# Autodesk Inventor assembly: BallBot
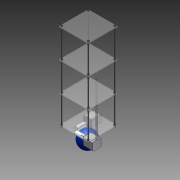
[picture p0: Inventor's stored thumbnail of the model, 180x180]
Saved by Autodesk Inventor 2012 (Build 160160000, 160)
## iProperties
Created: 2012-10-02
Part Number: BallBot
Document SubType Name: Assembly
Designer: agmlego
Author: agmlego
## Documents named in this file (8)
- C:\Users\Andrew G. Meyer\Documents\Projects\BallBot\Little\CAD\BallBot.iam
- C:\Users\Andrew G. Meyer\Documents\Projects\BallBot\Little\CAD\Platform.ipt
- C:\Users\Andrew G. Meyer\Documents\Projects\BallBot\Little\CAD\Rod.ipt
- C:\Users\Andrew G. Meyer\Documents\Projects\BallBot\Little\CAD\Ball.ipt
- C:\Users\Andrew G. Meyer\Documents\Inventor\Content Center Files\R2012\en-US\ANSI B 18.2.4.1 M(1)\ANSI B 18.2.4.1 M - M3 x 0.5Style 1.ipt
- C:\Users\Andrew G. Meyer\Documents\Projects\BallBot\Little\CAD\211-13-01.ipt
- C:\Users\Andrew G. Meyer\Documents\Projects\BallBot\Little\CAD\Roller.ipt
- C:\Users\Andrew G. Meyer\Documents\Inventor\Content Center Files\R2012\en-US\ANSI B18.3(08)\ANSI B18.3 - 4-48 UNF - 0.125(24).ipt
## Components (49 placed, 7 different names)
1. Platform:1 — Mate:50, Mate:51, Mate:53, Mate:55, Mate:80, Mate:81, Mate:82, Mate:83, Mate:84, Mate:85, Mate:86, Mate:87, Mate:95, Mate:96, Flush:9, Flush:10, Tangent:7, Flush:11, Flush:12
2. Platform:2 — Mate:34, Mate:35, Mate:36, Mate:37, Mate:56, Mate:57, Mate:58, Mate:59, Mate:60, Mate:61, Mate:62, Mate:63, Mate:89
3. Platform:3 — Mate:38, Mate:39, Mate:40, Mate:41, Mate:43, Mate:44, Mate:45, Mate:72, Mate:73, Mate:74, Mate:75, Mate:76, Mate:77, Mate:78, Mate:79, Mate:88
4. Platform:4 — Mate:42, Mate:64, Mate:65, Mate:66, Mate:67, Mate:68, Mate:69, Mate:70, Mate:71, Mate:88, Mate:89, Mate:90
5. Rod:1 — Mate:4, Mate:5, Mate:6, Mate:7, Mate:8, Mate:9, Mate:10, Mate:11, Mate:34, Mate:38, Mate:42, Mate:84, Flush:4, Flush:6
6. Rod:2 — Mate:1, Mate:3, Mate:12, Mate:13, Mate:14, Mate:15, Mate:16, Mate:17, Mate:35, Mate:39, Mate:43, Mate:80, Flush:1, Flush:5
7. Rod:3 — Mate:18, Mate:19, Mate:20, Mate:21, Mate:22, Mate:23, Mate:24, Mate:25, Mate:36, Mate:40, Mate:44, Mate:82, Flush:2, Flush:8, Mate:90
8. Rod:4 — Mate:26, Mate:27, Mate:28, Mate:29, Mate:30, Mate:31, Mate:32, Mate:33, Mate:37, Mate:41, Mate:45, Mate:86, Flush:3, Flush:7
9. Ball:1 — Tangent:5, Tangent:6, Tangent:7
10. Hex Nut Metric M3 x 0.5:1 — Mate:26, Mate:87, Flush:3
11. Hex Nut Metric M3 x 0.5:2 — Mate:27, Mate:55
12. Hex Nut Metric M3 x 0.5:3 — Mate:28, Mate:67
13. Hex Nut Metric M3 x 0.5:4 — Mate:29, Mate:63
14. Hex Nut Metric M3 x 0.5:5 — Mate:30, Mate:58
15. Hex Nut Metric M3 x 0.5:6 — Mate:31, Mate:78, Flush:7
16. Hex Nut Metric M3 x 0.5:7 — Mate:32, Mate:70
17. Hex Nut Metric M3 x 0.5:8 — Mate:33, Mate:74
18. Hex Nut Metric M3 x 0.5:9 — Mate:4, Mate:66
19. Hex Nut Metric M3 x 0.5:10 — Mate:5, Mate:57
20. Hex Nut Metric M3 x 0.5:11 — Mate:6, Mate:85, Flush:4
21. Hex Nut Metric M3 x 0.5:12 — Mate:7, Mate:53
22. Hex Nut Metric M3 x 0.5:13 — Mate:8, Mate:71
23. Hex Nut Metric M3 x 0.5:14 — Mate:9, Mate:75
24. Hex Nut Metric M3 x 0.5:15 — Mate:10, Mate:79, Flush:6
25. Hex Nut Metric M3 x 0.5:16 — Mate:11, Mate:62
26. Hex Nut Metric M3 x 0.5:17 — Mate:1, Mate:81, Flush:1
27. Hex Nut Metric M3 x 0.5:18 — Mate:3, Mate:51
28. Hex Nut Metric M3 x 0.5:19 — Mate:12, Mate:73
29. Hex Nut Metric M3 x 0.5:20 — Mate:13, Mate:56
30. Hex Nut Metric M3 x 0.5:21 — Mate:14, Mate:65
31. Hex Nut Metric M3 x 0.5:22 — Mate:15, Mate:69
32. Hex Nut Metric M3 x 0.5:23 — Mate:16, Mate:61
33. Hex Nut Metric M3 x 0.5:24 — Mate:17, Mate:77, Flush:5
34. Hex Nut Metric M3 x 0.5:25 — Mate:18, Mate:50
35. Hex Nut Metric M3 x 0.5:26 — Mate:19, Mate:60
36. Hex Nut Metric M3 x 0.5:27 — Mate:20, Mate:59
37. Hex Nut Metric M3 x 0.5:28 — Mate:21, Mate:68
38. Hex Nut Metric M3 x 0.5:29 — Mate:22, Mate:83, Flush:2
39. Hex Nut Metric M3 x 0.5:30 — Mate:23, Mate:76, Flush:8
40. Hex Nut Metric M3 x 0.5:31 — Mate:24, Mate:72
41. Hex Nut Metric M3 x 0.5:32 — Mate:25, Mate:64
42. 211-13-01:1 — Insert:1, Tangent:3, Tangent:4, Mate:95, Flush:10, Flush:11
43. 211-13-01:3 — Insert:2, Tangent:1, Tangent:2, Mate:96, Flush:9, Flush:12
44. Roller:1 — Insert:2, Mate:91, Mate:92, Tangent:6
45. Roller:2 — Insert:1, Mate:93, Mate:94, Tangent:5
46. Hexagon Socket Set Screw - Flat Point - Inch 4-48 UNF x 0.125:3 — Mate:91, Tangent:1
47. Hexagon Socket Set Screw - Flat Point - Inch 4-48 UNF x 0.125:1 — Mate:94, Tangent:4
48. Hexagon Socket Set Screw - Flat Point - Inch 4-48 UNF x 0.125:4 — Mate:92, Tangent:2
49. Hexagon Socket Set Screw - Flat Point - Inch 4-48 UNF x 0.125:2 — Mate:93, Tangent:3
## Relationships (110: Mate 89, Flush 12, Tangent 7, Insert 2)
- Mate:1: Rod:2 ↔ Hex Nut Metric M3 x 0.5:17
- Mate:3: Rod:2 ↔ Hex Nut Metric M3 x 0.5:18
- Mate:4: Rod:1 ↔ Hex Nut Metric M3 x 0.5:9
- Mate:5: Rod:1 ↔ Hex Nut Metric M3 x 0.5:10
- Mate:6: Rod:1 ↔ Hex Nut Metric M3 x 0.5:11
- Mate:7: Rod:1 ↔ Hex Nut Metric M3 x 0.5:12
- Mate:8: Rod:1 ↔ Hex Nut Metric M3 x 0.5:13
- Mate:9: Rod:1 ↔ Hex Nut Metric M3 x 0.5:14
- Mate:10: Rod:1 ↔ Hex Nut Metric M3 x 0.5:15
- Mate:11: Rod:1 ↔ Hex Nut Metric M3 x 0.5:16
- Mate:12: Rod:2 ↔ Hex Nut Metric M3 x 0.5:19
- Mate:13: Rod:2 ↔ Hex Nut Metric M3 x 0.5:20
- Mate:14: Rod:2 ↔ Hex Nut Metric M3 x 0.5:21
- Mate:15: Rod:2 ↔ Hex Nut Metric M3 x 0.5:22
- Mate:16: Rod:2 ↔ Hex Nut Metric M3 x 0.5:23
- Mate:17: Rod:2 ↔ Hex Nut Metric M3 x 0.5:24
- Mate:18: Rod:3 ↔ Hex Nut Metric M3 x 0.5:25
- Mate:19: Rod:3 ↔ Hex Nut Metric M3 x 0.5:26
- Mate:20: Rod:3 ↔ Hex Nut Metric M3 x 0.5:27
- Mate:21: Rod:3 ↔ Hex Nut Metric M3 x 0.5:28
- Mate:22: Rod:3 ↔ Hex Nut Metric M3 x 0.5:29
- Mate:23: Rod:3 ↔ Hex Nut Metric M3 x 0.5:30
- Mate:24: Rod:3 ↔ Hex Nut Metric M3 x 0.5:31
- Mate:25: Rod:3 ↔ Hex Nut Metric M3 x 0.5:32
- Mate:26: Rod:4 ↔ Hex Nut Metric M3 x 0.5:1
- Mate:27: Rod:4 ↔ Hex Nut Metric M3 x 0.5:2
- Mate:28: Rod:4 ↔ Hex Nut Metric M3 x 0.5:3
- Mate:29: Rod:4 ↔ Hex Nut Metric M3 x 0.5:4
- Mate:30: Rod:4 ↔ Hex Nut Metric M3 x 0.5:5
- Mate:31: Rod:4 ↔ Hex Nut Metric M3 x 0.5:6
- Mate:32: Rod:4 ↔ Hex Nut Metric M3 x 0.5:7
- Mate:33: Rod:4 ↔ Hex Nut Metric M3 x 0.5:8
- Mate:34: Platform:2 ↔ Rod:1
- Mate:35: Platform:2 ↔ Rod:2
- Mate:36: Platform:2 ↔ Rod:3
- Mate:37: Platform:2 ↔ Rod:4
- Mate:38: Platform:3 ↔ Rod:1
- Mate:39: Platform:3 ↔ Rod:2
- Mate:40: Platform:3 ↔ Rod:3
- Mate:41: Platform:3 ↔ Rod:4
- Mate:42: Platform:4 ↔ Rod:1
- Mate:43: Platform:3 ↔ Rod:2
- Mate:44: Platform:3 ↔ Rod:3
- Mate:45: Platform:3 ↔ Rod:4
- Mate:50: Platform:1 ↔ Hex Nut Metric M3 x 0.5:25
- Mate:51: Platform:1 ↔ Hex Nut Metric M3 x 0.5:18
- Mate:53: Platform:1 ↔ Hex Nut Metric M3 x 0.5:12
- Mate:55: Platform:1 ↔ Hex Nut Metric M3 x 0.5:2
- Mate:56: Platform:2 ↔ Hex Nut Metric M3 x 0.5:20
- Mate:57: Platform:2 ↔ Hex Nut Metric M3 x 0.5:10
- Mate:58: Platform:2 ↔ Hex Nut Metric M3 x 0.5:5
- Mate:59: Platform:2 ↔ Hex Nut Metric M3 x 0.5:27
- Mate:60: Platform:2 ↔ Hex Nut Metric M3 x 0.5:26
- Mate:61: Platform:2 ↔ Hex Nut Metric M3 x 0.5:23
- Mate:62: Platform:2 ↔ Hex Nut Metric M3 x 0.5:16
- Mate:63: Platform:2 ↔ Hex Nut Metric M3 x 0.5:4
- Mate:64: Platform:4 ↔ Hex Nut Metric M3 x 0.5:32
- Mate:65: Platform:4 ↔ Hex Nut Metric M3 x 0.5:21
- Mate:66: Platform:4 ↔ Hex Nut Metric M3 x 0.5:9
- Mate:67: Platform:4 ↔ Hex Nut Metric M3 x 0.5:3
- Mate:68: Platform:4 ↔ Hex Nut Metric M3 x 0.5:28
- Mate:69: Platform:4 ↔ Hex Nut Metric M3 x 0.5:22
- Mate:70: Platform:4 ↔ Hex Nut Metric M3 x 0.5:7
- Mate:71: Platform:4 ↔ Hex Nut Metric M3 x 0.5:13
- Mate:72: Platform:3 ↔ Hex Nut Metric M3 x 0.5:31
- Mate:73: Platform:3 ↔ Hex Nut Metric M3 x 0.5:19
- Mate:74: Platform:3 ↔ Hex Nut Metric M3 x 0.5:8
- Mate:75: Platform:3 ↔ Hex Nut Metric M3 x 0.5:14
- Mate:76: Platform:3 ↔ Hex Nut Metric M3 x 0.5:30
- Mate:77: Platform:3 ↔ Hex Nut Metric M3 x 0.5:24
- Mate:78: Platform:3 ↔ Hex Nut Metric M3 x 0.5:6
- Mate:79: Platform:3 ↔ Hex Nut Metric M3 x 0.5:15
- Mate:80: Platform:1 ↔ Rod:2
- Mate:81: Platform:1 ↔ Hex Nut Metric M3 x 0.5:17
- Mate:82: Platform:1 ↔ Rod:3
- Mate:83: Platform:1 ↔ Hex Nut Metric M3 x 0.5:29
- Mate:84: Platform:1 ↔ Rod:1
- Mate:85: Platform:1 ↔ Hex Nut Metric M3 x 0.5:11
- Mate:86: Platform:1 ↔ Rod:4
- Mate:87: Platform:1 ↔ Hex Nut Metric M3 x 0.5:1
- Flush:1 (-1 mm): Rod:2 ↔ Hex Nut Metric M3 x 0.5:17
- Flush:2 (-1 mm): Rod:3 ↔ Hex Nut Metric M3 x 0.5:29
- Flush:3 (-1 mm): Rod:4 ↔ Hex Nut Metric M3 x 0.5:1
- Flush:4 (-1 mm): Rod:1 ↔ Hex Nut Metric M3 x 0.5:11
- Flush:5 (-1 mm): Rod:2 ↔ Hex Nut Metric M3 x 0.5:24
- Flush:6 (-1 mm): Rod:1 ↔ Hex Nut Metric M3 x 0.5:15
- Flush:7 (-1 mm): Rod:4 ↔ Hex Nut Metric M3 x 0.5:6
- Flush:8 (-1 mm): Rod:3 ↔ Hex Nut Metric M3 x 0.5:30
- Mate:88 (95 mm): Platform:3 ↔ Platform:4
- Mate:89 (95 mm): Platform:2 ↔ Platform:4
- Mate:90: Platform:4 ↔ Rod:3
- Insert:1: 211-13-01:1 ↔ Roller:2
- Insert:2: 211-13-01:3 ↔ Roller:1
- Mate:91: Roller:1 ↔ Hexagon Socket Set Screw - Flat Point - Inch 4-48 UNF x 0.125:3
- Mate:92: Roller:1 ↔ Hexagon Socket Set Screw - Flat Point - Inch 4-48 UNF x 0.125:4
- Mate:93: Roller:2 ↔ Hexagon Socket Set Screw - Flat Point - Inch 4-48 UNF x 0.125:2
- Mate:94: Roller:2 ↔ Hexagon Socket Set Screw - Flat Point - Inch 4-48 UNF x 0.125:1
- Tangent:1: 211-13-01:3 ↔ Hexagon Socket Set Screw - Flat Point - Inch 4-48 UNF x 0.125:3
- Tangent:2: 211-13-01:3 ↔ Hexagon Socket Set Screw - Flat Point - Inch 4-48 UNF x 0.125:4
- Tangent:3: 211-13-01:1 ↔ Hexagon Socket Set Screw - Flat Point - Inch 4-48 UNF x 0.125:2
- Tangent:4: 211-13-01:1 ↔ Hexagon Socket Set Screw - Flat Point - Inch 4-48 UNF x 0.125:1
- Tangent:5: Ball:1 ↔ Roller:2
- Tangent:6: Ball:1 ↔ Roller:1
- Mate:95: Platform:1 ↔ 211-13-01:1
- Mate:96: Platform:1 ↔ 211-13-01:3
- Flush:9 (10 mm): Platform:1 ↔ 211-13-01:3
- Flush:10 (10 mm): Platform:1 ↔ 211-13-01:1
- Tangent:7 (10 mm): Platform:1 ↔ Ball:1
- Flush:11 (-6 mm): Platform:1 ↔ 211-13-01:1
- Flush:12 (-6 mm): Platform:1 ↔ 211-13-01:3
